# Autodesk Inventor assembly: Fr.wing_assy
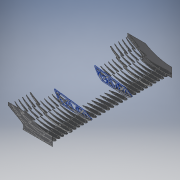
[picture p0: Inventor's stored thumbnail of the model, 180x180]
Saved by Autodesk Inventor 2018.2 (Build 222227000, 227)
## iProperties
Created: 2018-03-05
Part Number: Fr.wing_assy
Material: 一般
Document SubType Name: Assembly
Designer: ku_sk
Author: ku_sk
## Documents named in this file (8)
- C:\Users\ku_sk\Documents\Inventor\Aero\KS-15\Fr.wing\Fr.wing_assy.iam
- C:\Users\ku_sk\Documents\Inventor\Aero\KS-15\Fr.wing\parts\mainflap_side\mainflap_side.iam
- C:\Users\ku_sk\Documents\Inventor\Aero\KS-15\Fr.wing\parts\mainflap_center\mainflap_center.iam
- C:\Users\ku_sk\Documents\Inventor\Aero\KS-15\Fr.wing\parts\subflap\subflap.iam
- C:\Users\ku_sk\Documents\Inventor\Aero\KS-15\Fr.wing\parts\bracket1\bracket1.ipt
- C:\Users\ku_sk\Documents\Inventor\Aero\KS-15\Fr.wing\parts\bracket2.ipt
- C:\Users\ku_sk\Documents\Inventor\Aero\KS-15\Fr.wing\parts\endplate.ipt
- C:\Users\ku_sk\Documents\Inventor\Aero\KS-15\Fr.wing\parts\endplate1.ipt
## Components (17 placed, 7 different names)
1. mainflap_center:1 [sub-assembly] — フラッシュ:1, メイト:1, メイト:2, メイト:3, メイト:4, メイト:5, メイト:6, メイト:7, 角度:1
2. mainflap_side:1 [sub-assembly] — メイト:2, メイト:4, メイト:7, メイト:8, メイト:9, メイト:10, フラッシュ:2, メイト:46
3. mainflap_side:2 [sub-assembly] — メイト:3, メイト:5, メイト:6, メイト:11, メイト:12, メイト:13, フラッシュ:4, メイト:49
4. mainflap_side:3 [sub-assembly] — メイト:8, メイト:9, メイト:10, フラッシュ:3, メイト:45
5. mainflap_side:4 [sub-assembly] — メイト:11, メイト:12, メイト:13, フラッシュ:5, メイト:44
6. subflap:1 [sub-assembly] — メイト:14, メイト:15, メイト:19, フラッシュ:2, メイト:20, メイト:21
7. subflap:2 [sub-assembly] — メイト:14, メイト:15, メイト:19, フラッシュ:3, フラッシュ:7
8. subflap:3 [sub-assembly] — メイト:22, メイト:23, フラッシュ:7
9. subflap:4 [sub-assembly] — メイト:16, メイト:17, メイト:18, フラッシュ:4, メイト:20, メイト:21
10. subflap:5 [sub-assembly] — メイト:16, メイト:17, メイト:18, フラッシュ:5, フラッシュ:6
11. subflap:6 [sub-assembly] — メイト:22, メイト:23, フラッシュ:6
12. endplate:1 — メイト:44, フラッシュ:8, フラッシュ:9
13. endplate1:1 — メイト:45, フラッシュ:8, フラッシュ:9
14. bracket2:1 — メイト:46
15. bracket2:2 — メイト:49
16. bracket1:1
17. bracket1:2
## Relationships (37: Mate 27, Flush 9, Angle 1)
- フラッシュ:1 [Flush]: mainflap_center:1
- メイト:1 [Mate]: mainflap_center:1
- メイト:2 [Mate] (4 mm): mainflap_center:1 ↔ mainflap_side:1
- メイト:3 [Mate] (4 mm): mainflap_center:1 ↔ mainflap_side:2
- メイト:4 [Mate]: mainflap_center:1 ↔ mainflap_side:1
- メイト:5 [Mate]: mainflap_center:1 ↔ mainflap_side:2
- メイト:6 [Mate]: mainflap_center:1 ↔ mainflap_side:2
- メイト:7 [Mate]: mainflap_center:1 ↔ mainflap_side:1
- メイト:8 [Mate] (4 mm): mainflap_side:1 ↔ mainflap_side:3
- メイト:9 [Mate]: mainflap_side:1 ↔ mainflap_side:3
- メイト:10 [Mate]: mainflap_side:1 ↔ mainflap_side:3
- メイト:11 [Mate] (4 mm): mainflap_side:2 ↔ mainflap_side:4
- メイト:12 [Mate]: mainflap_side:2 ↔ mainflap_side:4
- メイト:13 [Mate]: mainflap_side:2 ↔ mainflap_side:4
- メイト:14 [Mate]: subflap:1 ↔ subflap:2
- メイト:15 [Mate]: subflap:1 ↔ subflap:2
- メイト:16 [Mate] (4 mm): subflap:4 ↔ subflap:5
- メイト:17 [Mate]: subflap:4 ↔ subflap:5
- メイト:18 [Mate]: subflap:4 ↔ subflap:5
- メイト:19 [Mate] (4 mm): subflap:1 ↔ subflap:2
- フラッシュ:2 [Flush]: mainflap_side:1 ↔ subflap:1
- フラッシュ:3 [Flush]: mainflap_side:3 ↔ subflap:2
- フラッシュ:4 [Flush]: mainflap_side:2 ↔ subflap:4
- フラッシュ:5 [Flush]: mainflap_side:4 ↔ subflap:5
- メイト:20 [Mate]: subflap:1 ↔ subflap:4
- メイト:21 [Mate]: subflap:1 ↔ subflap:4
- メイト:22 [Mate]: subflap:3 ↔ subflap:6
- メイト:23 [Mate]: subflap:3 ↔ subflap:6
- フラッシュ:6 [Flush]: subflap:5 ↔ subflap:6
- フラッシュ:7 [Flush]: subflap:2 ↔ subflap:3
- メイト:44 [Mate]: mainflap_side:4 ↔ endplate:1
- メイト:45 [Mate]: mainflap_side:3 ↔ endplate1:1
- フラッシュ:8 [Flush]: endplate:1 ↔ endplate1:1
- フラッシュ:9 [Flush]: endplate:1 ↔ endplate1:1
- 角度:1 [Angle] (2 deg): mainflap_center:1
- メイト:46 [Mate]: mainflap_side:1 ↔ bracket2:1
- メイト:49 [Mate]: mainflap_side:2 ↔ bracket2:2
